# Autodesk Inventor assembly: robot
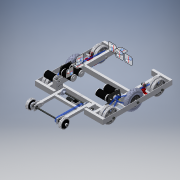
[picture p0: Inventor's stored thumbnail of the model, 180x180]
Saved by Autodesk Inventor 2016 (Build 200138000, 138)
## iProperties
Created: 2016-01-18
Part Number: robot
Document SubType Name: Assembly
Designer: gus
Mass: 20725.8 g
Surface Area: 42338.2 cm^2
Volume: 8952.51 cm^3
Density: 2.31508 g/cm^3
Author: gus
## Documents named in this file (4)
- \\Mac\Home\Desktop\2016 robot cad\robot.iam
- \\Mac\Home\Desktop\2016 robot cad\chassis\chassis.iam
- \\Mac\Home\Desktop\2016 robot cad\roller wheels\roller wheels.iam
- \\Mac\Home\Desktop\2016 robot cad\chassis\chain tensioner\chain tensioner.iam
## Components (4 placed, 3 different names)
1. chassis:1 [sub-assembly] — Cylindrical:1, Mate:1, Mate:2, Flush:1, Mate:3, Flush:2
2. roller wheels:1 [sub-assembly] — Cylindrical:1, Mate:1
3. chain tensioner:1 [sub-assembly] — Mate:2, Flush:1
4. chain tensioner:2 [sub-assembly] — Mate:3, Flush:2
## Relationships (6: Mate 3, Flush 2, CylindricalJoint 1)
- Cylindrical:1: chassis:1 ↔ roller wheels:1
- Mate:1 (10.16 mm): chassis:1 ↔ roller wheels:1
- Mate:2: chassis:1 ↔ chain tensioner:1
- Flush:1: chassis:1 ↔ chain tensioner:1
- Mate:3: chassis:1 ↔ chain tensioner:2
- Flush:2: chassis:1 ↔ chain tensioner:2
